# Autodesk Inventor assembly: EL2-C-100
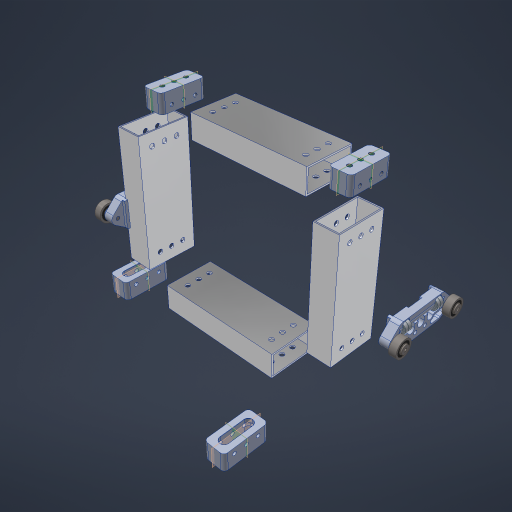
[picture p0: Inventor's stored thumbnail of the model, 512x512]
Saved by Autodesk Inventor 2023.4 (Build 274418000, 418)
## iProperties
Created: 2025-01-11
Part Number: EL2-C-100
Document SubType Name: Assembly
Designer: brand
Author: brand
## Documents named in this file (4)
- C:\Users\brand\OneDrive\Documents\GitHub\robotics 23\2025-ReefScape---CAD\Elevator\EL2\EL2-C-100.iam
- C:\Users\brand\OneDrive\Documents\GitHub\robotics 23\2025-ReefScape---CAD\Elevator\EL2\EL2-C-001.ipt
- C:\Users\brand\OneDrive\Documents\GitHub\robotics 23\2025-ReefScape---CAD\COMMON PARTS\WCP Elevator parts\WCP-0897\WCP-0897.iam
- C:\Users\brand\OneDrive\Documents\GitHub\robotics 23\2025-ReefScape---CAD\Elevator\EL2\EL2-005.ipt
## Components (10 placed, 3 different names)
1. EL2-C-001:1
2. EL2-C-001:2 — Mate:1, Mate:2
3. EL2-C-001:3
4. EL2-C-001:4
5. WCP-0897:1 [sub-assembly]
6. WCP-0897:2 [sub-assembly] — Mate:1, Mate:2
7. EL2-005:1
8. EL2-005:2
9. EL2-005:3
10. EL2-005:4
## Relationships (2: Mate 2)
- Mate:1: EL2-C-001:2 ↔ WCP-0897:2
- Mate:2: EL2-C-001:2 ↔ WCP-0897:2
